# Autodesk Inventor assembly: ensamble_pcb
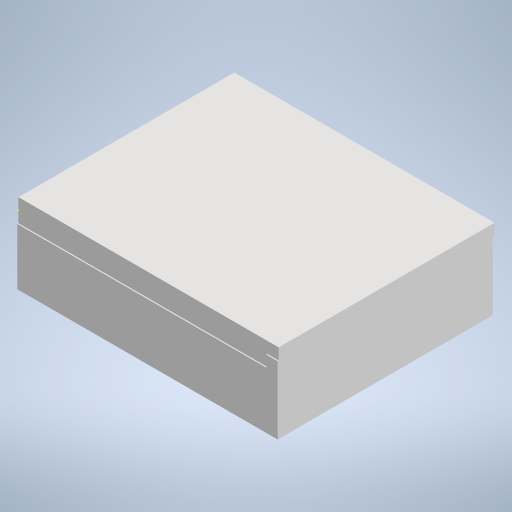
[picture p0: Inventor's stored thumbnail of the model, 512x512]
Saved by Autodesk Inventor 2024.3 (Build 283343000, 343)
## iProperties
Created: 2025-07-17
Part Number: ensamble_pcb
Document SubType Name: Assembly
Designer: Damian
Author: Damian
## Documents named in this file (3)
- D:\Damian\Utal\Memoria_clino\Memoria-clinostato\Inventor\Diseño_caja\Diseño_lp8_bme\ensamble_pcb.iam
- D:\Damian\Utal\Memoria_clino\Memoria-clinostato\Inventor\Diseño_caja\Diseño_lp8_bme\carcasa_pcb.ipt
- D:\Damian\Utal\Memoria_clino\Memoria-clinostato\Inventor\Diseño_caja\Diseño_lp8_bme\tapa_pcb.ipt
## Components (2 placed, 2 different names)
1. carcasa_pcb:1 — Coincidencia:1, Coincidencia:2, Coincidencia:3, Coincidencia:4, Coincidencia:5
2. tapa_pcb:1 — Coincidencia:4, Coincidencia:5
## Relationships (5: Mate 5)
- Coincidencia:1 [Mate]: carcasa_pcb:1
- Coincidencia:2 [Mate]: carcasa_pcb:1
- Coincidencia:3 [Mate]: carcasa_pcb:1
- Coincidencia:4 [Mate]: carcasa_pcb:1 ↔ tapa_pcb:1
- Coincidencia:5 [Mate]: carcasa_pcb:1 ↔ tapa_pcb:1
